# Autodesk Inventor assembly: Wheel Insert Test Fit
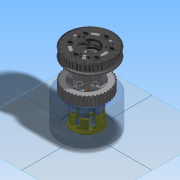
[picture p0: Inventor's stored thumbnail of the model, 180x180]
Saved by Autodesk Inventor 2014 SP2 (Build 180246200, 246)
## iProperties
Created: 2014-05-22
Part Number: Wheel Insert Test Fit
Document SubType Name: Assembly
Designer: dliu
Author: dliu
## Documents named in this file (5)
- C:\Users\dliu\Dropbox\dbhome\electric-longboard\dliu\Wheel Insert\Wheel Insert Test Fit.iam
- C:\Users\dliu\Dropbox\dbhome\electric-longboard\dliu\Board\Wheel Blank Pro 83mm.ipt
- C:\Users\dliu\Dropbox\dbhome\electric-longboard\dliu\Wheel Insert\Wheel Insert Retainer.ipt
- C:\Users\dliu\Dropbox\dbhome\electric-longboard\dliu\Wheel Insert\Wheel Insert Inner.ipt
- C:\Users\dliu\Dropbox\dbhome\electric-longboard\dliu\Wheel Insert\Wheel Insert InnerAdapter Context.iam
## Components (4 placed, 4 different names)
1. Wheel Blank Pro 83mm:1
2. Wheel Insert Retainer:1 — Mate:1, Mate:2, Mate:5
3. Wheel Insert Inner:1 — Mate:4, Mate:5
4. Wheel Insert InnerAdapter Context:1 [sub-assembly]
## Relationships (4: Mate 4)
- Mate:1: Wheel Insert Retainer:1
- Mate:2: Wheel Insert Retainer:1
- Mate:4: Wheel Insert Inner:1
- Mate:5: Wheel Insert Retainer:1 ↔ Wheel Insert Inner:1
